# Autodesk Inventor assembly: PIHTI-for-Boron
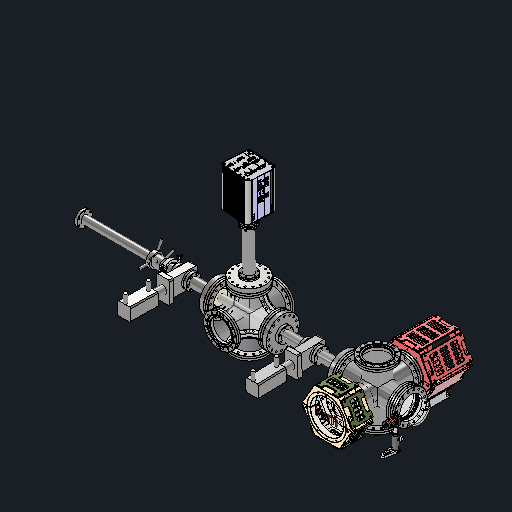
[picture p0: Inventor's stored thumbnail of the model, 512x512]
Saved by Autodesk Inventor 2027.1 (Build 311270010, 270A)
## iProperties
Created: 2024-05-09
Part Number: PIHTI-for-Boron
Document SubType Name: Assembly
Designer: kuzmin
Mass: 19614.5 g
Surface Area: 13609.5 cm^2
Volume: 3689.47 cm^3
Density: 5.31636 g/cm^3
Author: kuzmin
## Documents named in this file (25)
- C:\Users\queezz\Dropbox\Drawings\pihti-cad\Plasma Vessel\PIHTI-for-Boron.iam
- C:\Users\queezz\Dropbox\Drawings\pihti-cad\Plasma Vessel\Plasma-vacuum-cross\Plasma-vacuum-vessel-152IC-cross.iam
- C:\Users\queezz\Dropbox\Drawings\pihti-cad\Plasma Vessel\Plasma-Flange-2024\cathode-box-on-a-flange.iam
- C:\Users\queezz\Dropbox\Drawings\pihti-cad\Plasma Vessel\Cathode-Flange-Cage\CathodeCage.iam
- C:\Users\queezz\Dropbox\Drawings\pihti-cad\Plasma Vessel\Cathode-Anode-Flange\Cathode-Anode-70IC-flange-with-feeds.iam
- C:\Users\queezz\Dropbox\Drawings\pihti-cad\Plasma Vessel\Plasma-Box\Plasma-box-hayashi-aka-upgrade.iam
- C:\Users\queezz\Dropbox\Drawings\pihti-cad\ContentCenter\Fastners\M3x8-SHCS.ipt
- C:\Users\queezz\Dropbox\Drawings\pihti-cad\Plasma Vessel\Plasma-Box\probe-gate-with-spindel.iam
- C:\Users\queezz\Dropbox\Drawings\pihti-cad\Plasma Vessel\Cathode-Anode-Flange\cf70_spacer.ipt
- C:\Users\queezz\Dropbox\Drawings\pihti-cad\Plasma Vessel\Plasma-Box\anode-on-flange.iam
- C:\Users\queezz\Dropbox\Drawings\pihti-cad\Plasma Vessel\entrance-mesh-assembly.iam
- C:\Users\queezz\Dropbox\Drawings\pihti-cad\Plasma Vessel\Oring-probe-flange-with-GV.iam
- C:\Users\queezz\Dropbox\Drawings\pihti-cad\Plasma Vessel\Plasma-Box-Support.ipt
- C:\Users\queezz\Dropbox\Drawings\pihti-cad\Plasma Vessel\probe-port-mesh-welded.iam
- C:\Users\queezz\Dropbox\Drawings\pihti-cad\Plasma Vessel\Mesh-mounting-help.ipt
- C:\Users\queezz\Dropbox\Drawings\pihti-cad\Plasma Vessel\Cathode-Flange-Cage\Short-Cage.iam
- C:\Users\queezz\Dropbox\Drawings\pihti-cad\ContentCenter\CF-parts\CF-Flanges\CF_152-70.ipt
- C:\Users\queezz\Dropbox\Drawings\pihti-cad\ContentCenter\CF-parts\CF70-nipple\CF70-nipple.iam
- C:\Users\queezz\Dropbox\Drawings\pihti-cad\ContentCenter\CF-parts\CF70-gate-valve\Gatevalve_70_pneumatic.iam
- C:\Users\queezz\Dropbox\Drawings\pihti-cad\BoronProbe\BoronProbe.iam
- C:\Users\queezz\Dropbox\Drawings\pihti-cad\ContentCenter\ulvac\Qulee_BGM2-102_202.ipt
- C:\Users\queezz\Dropbox\Drawings\pihti-cad\Plasma Vessel\Plasma-vacuum-cross\UFC-152.ipt
- C:\Users\queez\Dropbox\Drawings\PIHTI\Plasma Vessel\Plasma-vacuum-cross\UFC.ipt
- C:\Users\queezz\Dropbox\Drawings\pihti-cad\BoronProbe\GlassPort-idea.ipt
- C:\Users\queezz\Dropbox\Drawings\pihti-cad\ContentCenter\Optics\collimator.iam
## Components (34 placed, 23 different names)
1. Plasma-vacuum-vessel-152IC-cross:1 [sub-assembly] — Mate:1, Flush:1, Flush:2, Rotational:1, Mate:15, Mate:16, Rigid:17, Rigid:18, Mate:21, Rotational:21, Flush:4
2. cathode-box-on-a-flange:1 [sub-assembly] — Rotational:1, Rotational:2, Mate:2, Mate:5, Rigid:10
3. CathodeCage:1 [sub-assembly] — Rotational:2
4. Cathode-Anode-70IC-flange-with-feeds:1 [sub-assembly] — Mate:2, Mate:5, Mate:6
5. Plasma-box-hayashi-aka-upgrade:1 [sub-assembly] — Mate:3, Mate:4, Hinge Angle, Mate:7, Mate:8, Mate:9, Mate:13, Mate:17
6. probe-gate-with-spindel:1 [sub-assembly] — Mate:3, Mate:4, Hinge Angle
7. cf70_spacer:1 — Rigid:10, Mate:6
8. anode-on-flange:1 [sub-assembly] — Mate:7, Mate:8, Mate:9, Rigid:11, Rigid:12, Rigid:13, Rigid:14
9. entrance-mesh-assembly:1 [sub-assembly] — Mate:13, Mate:17, Mate:19
10. Oring-probe-flange-with-GV:1 [sub-assembly] — Mate:15, Rigid:16, Rotational:3
11. Plasma-Box-Support:1 — Mate:16, Flush:3
12. probe-port-mesh-welded:1 [sub-assembly] — Mate:19
13. Mesh-mounting-help:1 — Rigid:16
14. Short-Cage:1 [sub-assembly] — Rigid:17
15. Plasma-vacuum-vessel-152IC-cross:2 [sub-assembly] — Rotational:20, Rotational:3, Rigid:25
16. CF_152-70:1 — Rigid:18, Mate:20, Rigid:21
17. CF_152-70:2 — Rotational:20, Mate:20, Rigid:24
18. CF70-nipple:1 [sub-assembly] — Rigid:21, Rigid:22
19. CF70-nipple:2 [sub-assembly] — Rigid:23, Rigid:24
20. Gatevalve_70_pneumatic:1 [sub-assembly] — Rigid:22, Rigid:23
21. BoronProbe:1 [sub-assembly] — Mate:21
22. CF_152-70:3 — Rigid:25, Rotational:4
23. Qulee_BGM2-102_202:1 — Rotational:4
24. UFC-152:1 — Rotational:21, Rigid:26
25. GlassPort-idea:1 — Rigid:26
26. collimator:1 [sub-assembly] — Flush:4
27. SS ISO 4762 M3 x 8:5 — Rigid:11
28. SS ISO 4762 M3 x 8:6 — Rigid:12
29. SS ISO 4762 M3 x 8:7 — Rigid:14
30. SS ISO 4762 M3 x 8:8 — Rigid:13
31. SS ISO 4762 M3 x 8:1
32. SS ISO 4762 M3 x 8:2
33. SS ISO 4762 M3 x 8:3
34. SS ISO 4762 M3 x 8:4
## Relationships (42: Mate 17, WeldJoint 14, RevoluteJoint 6, Flush 4, Angle 1)
- Mate:1: Plasma-vacuum-vessel-152IC-cross:1
- Flush:1: Plasma-vacuum-vessel-152IC-cross:1
- Flush:2: Plasma-vacuum-vessel-152IC-cross:1
- Rotational:1 [RevoluteJoint]: Plasma-vacuum-vessel-152IC-cross:1 ↔ cathode-box-on-a-flange:1
- Rotational:2 [RevoluteJoint]: cathode-box-on-a-flange:1 ↔ CathodeCage:1
- Mate:2: cathode-box-on-a-flange:1 ↔ Cathode-Anode-70IC-flange-with-feeds:1
- Mate:3: Plasma-box-hayashi-aka-upgrade:1 ↔ probe-gate-with-spindel:1
- Mate:4: Plasma-box-hayashi-aka-upgrade:1 ↔ probe-gate-with-spindel:1
- Hinge Angle [Angle] (45 deg): Plasma-box-hayashi-aka-upgrade:1 ↔ probe-gate-with-spindel:1
- Mate:5: cathode-box-on-a-flange:1 ↔ Cathode-Anode-70IC-flange-with-feeds:1
- Rigid:10 [WeldJoint]: cathode-box-on-a-flange:1 ↔ cf70_spacer:1
- Mate:6: Cathode-Anode-70IC-flange-with-feeds:1 ↔ cf70_spacer:1
- Mate:7: Plasma-box-hayashi-aka-upgrade:1 ↔ anode-on-flange:1
- Mate:8: Plasma-box-hayashi-aka-upgrade:1 ↔ anode-on-flange:1
- Mate:9: Plasma-box-hayashi-aka-upgrade:1 ↔ anode-on-flange:1
- Rigid:11 [WeldJoint]: anode-on-flange:1 ↔ SS ISO 4762 M3 x 8:5
- Rigid:12 [WeldJoint]: anode-on-flange:1 ↔ SS ISO 4762 M3 x 8:6
- Rigid:13 [WeldJoint]: anode-on-flange:1 ↔ SS ISO 4762 M3 x 8:8
- Rigid:14 [WeldJoint]: anode-on-flange:1 ↔ SS ISO 4762 M3 x 8:7
- [Mate]: Plasma-vacuum-vessel-152IC-cross:1 ↔ Oring-probe-flange-with-GV:1
- Mate:13: Plasma-box-hayashi-aka-upgrade:1 ↔ entrance-mesh-assembly:1
- Mate:15: Plasma-vacuum-vessel-152IC-cross:1 ↔ Oring-probe-flange-with-GV:1
- Mate:16: Plasma-vacuum-vessel-152IC-cross:1 ↔ Plasma-Box-Support:1
- Flush:3: Plasma-Box-Support:1
- Mate:17: Plasma-box-hayashi-aka-upgrade:1 ↔ entrance-mesh-assembly:1
- Rigid:16 [WeldJoint]: Oring-probe-flange-with-GV:1 ↔ Mesh-mounting-help:1
- Rigid:17 [WeldJoint]: Plasma-vacuum-vessel-152IC-cross:1 ↔ Short-Cage:1
- Mate:19: entrance-mesh-assembly:1 ↔ probe-port-mesh-welded:1
- Rigid:18 [WeldJoint]: Plasma-vacuum-vessel-152IC-cross:1 ↔ CF_152-70:1
- Rotational:20 [RevoluteJoint]: Plasma-vacuum-vessel-152IC-cross:2 ↔ CF_152-70:2
- Mate:20: CF_152-70:1 ↔ CF_152-70:2
- Rotational:3 [RevoluteJoint]: Oring-probe-flange-with-GV:1 ↔ Plasma-vacuum-vessel-152IC-cross:2
- Rigid:21 [WeldJoint]: CF_152-70:1 ↔ CF70-nipple:1
- Rigid:22 [WeldJoint]: CF70-nipple:1 ↔ Gatevalve_70_pneumatic:1
- Rigid:23 [WeldJoint]: CF70-nipple:2 ↔ Gatevalve_70_pneumatic:1
- Rigid:24 [WeldJoint]: CF_152-70:2 ↔ CF70-nipple:2
- Mate:21: Plasma-vacuum-vessel-152IC-cross:1 ↔ BoronProbe:1
- Rigid:25 [WeldJoint]: Plasma-vacuum-vessel-152IC-cross:2 ↔ CF_152-70:3
- Rotational:4 [RevoluteJoint]: CF_152-70:3 ↔ Qulee_BGM2-102_202:1
- Rotational:21 [RevoluteJoint]: Plasma-vacuum-vessel-152IC-cross:1 ↔ UFC-152:1
- Rigid:26 [WeldJoint]: UFC-152:1 ↔ GlassPort-idea:1
- Flush:4 (20 mm): Plasma-vacuum-vessel-152IC-cross:1 ↔ collimator:1
